# Autodesk Inventor assembly: Ring Funnel
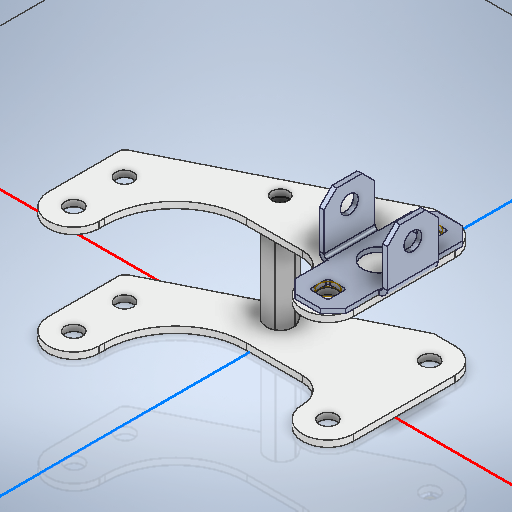
[picture p0: Inventor's stored thumbnail of the model, 512x512]
Saved by Autodesk Inventor 2026 (Build 300175000, 175)
## iProperties
Created: 2025-04-05
Part Number: Ring Funnel
Document SubType Name: Assembly
Designer: avere
Author: avere
## Documents named in this file (5)
- C:\Users\avere\OneDrive\Documents\VEX-CAD\V5-CAD\Drivetrain\Drivebay Right\Ring Funnel.iam
- C:\Users\avere\OneDrive\Documents\VEX-CAD\V5-CAD\Drivetrain\Drivebay Right\Front Gusset.ipt
- C:\Users\avere\OneDrive\Documents\VEX-CAD\VEX-CAD-Inventor\Structure\Standoff\Standoff 1.00.ipt
- C:\Users\avere\OneDrive\Documents\VEX-CAD\VEX-CAD-Inventor\Structure\Standoff.ipt
- C:\Users\avere\OneDrive\Documents\VEX-CAD\VEX-CAD-Inventor\Motion\Pneumatics\Legacy - SMC Pneumatics\Cylinder Rod Pivot.ipt
## Components (4 placed, 3 different names)
1. Front Gusset:1 — Mate:2, Insert:1, Insert:2, Mate:1
2. Front Gusset:2 — Mate:2, Insert:3
3. Standoff 1.00:1 — Insert:3, Insert:1
4. Cylinder Rod Pivot:1 — Insert:2, Mate:1
## Relationships (5: Insert 3, Mate 2)
- Mate:2: Front Gusset:1 ↔ Front Gusset:2
- Insert:3: Front Gusset:2 ↔ Standoff 1.00:1
- Insert:1: Front Gusset:1 ↔ Standoff 1.00:1
- Insert:2: Front Gusset:1 ↔ Cylinder Rod Pivot:1
- Mate:1: Front Gusset:1 ↔ Cylinder Rod Pivot:1
